# Autodesk Inventor assembly: carkifelek-ass
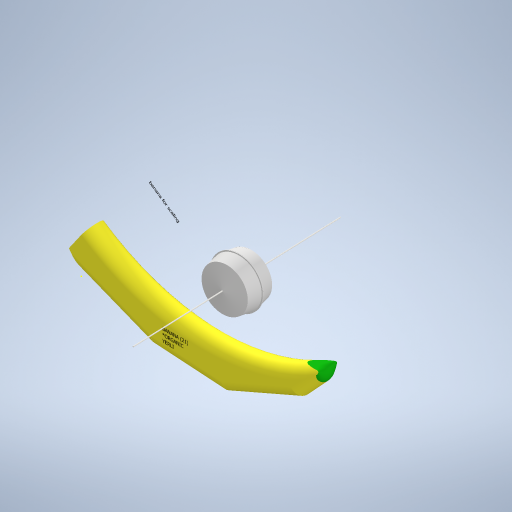
[picture p0: Inventor's stored thumbnail of the model, 512x512]
Saved by Autodesk Inventor 2023.2 (Build 272271000, 271)
## iProperties
Created: 2023-03-22
Part Number: carkifelek-ass
Document SubType Name: Assembly
Designer: sarp1
Author: sarp1
## Documents named in this file (7)
- C:\Users\sarp1\Documents\carkifelek-final\carkifelek-ass.iam
- C:\Users\sarp1\Documents\carkifelek-final\carkifelek-ass\Design Accelerator\Spur Gears1.iam
- C:\Users\sarp1\Documents\carkifelek-final\carkifelek-ass\Design Accelerator\Spur Gear11.ipt
- C:\Users\sarp1\Documents\carkifelek-final\dondurgec.ipt
- C:\Users\sarp1\Documents\carkifelek-final\carkifelek-ass\Design Accelerator\Spur Gear21.ipt
- C:\Users\sarp1\Documents\carkifelek-final\kab.ipt
- C:\Users\sarp1\Documents\carkifelek-final\scale.ipt
## Components (12 placed, 6 different names)
1. carks:1 [sub-assembly]
2. kucuk:1 — Cylindrical:2, Mate:5
3. dondurgec:1 — Cylindrical:1, Mate:1, Cylindrical:2, Cylindrical:3, Cylindrical:4, Cylindrical:5, Mate:3, Mate:4
4. boyuk:1 — Cylindrical:1, Mate:1, Cylindrical:11
5. kucuk:2 — Cylindrical:3, Mate:4
6. kucuk:3 — Cylindrical:4, Mate:3, Cylindrical:7
7. kucuk:4 — Cylindrical:5, Cylindrical:8, Mate:6
8. dondurgec:2 — Cylindrical:6, Mate:2, Cylindrical:7, Cylindrical:8, Mate:5, Mate:6
9. boyuk:2 — Cylindrical:6, Mate:2, Cylindrical:9, Cylindrical:10
10. kab:1 — Cylindrical:9, Cylindrical:10, Mate:7
11. kab:2 — Cylindrical:11, Mate:7
12. scale:1
## Relationships (18: CylindricalJoint 11, Mate 7)
- Cylindrical:1: dondurgec:1 ↔ boyuk:1
- Mate:1: dondurgec:1 ↔ boyuk:1
- Cylindrical:2: kucuk:1 ↔ dondurgec:1
- Cylindrical:3: dondurgec:1 ↔ kucuk:2
- Cylindrical:4: dondurgec:1 ↔ kucuk:3
- Cylindrical:5: dondurgec:1 ↔ kucuk:4
- Cylindrical:6: dondurgec:2 ↔ boyuk:2
- Mate:2: dondurgec:2 ↔ boyuk:2
- Mate:3: dondurgec:1 ↔ kucuk:3
- Mate:4: dondurgec:1 ↔ kucuk:2
- Cylindrical:7: kucuk:3 ↔ dondurgec:2
- Cylindrical:8: kucuk:4 ↔ dondurgec:2
- Mate:5: kucuk:1 ↔ dondurgec:2
- Mate:6: kucuk:4 ↔ dondurgec:2
- Cylindrical:9: boyuk:2 ↔ kab:1
- Cylindrical:10: boyuk:2 ↔ kab:1
- Cylindrical:11: boyuk:1 ↔ kab:2
- Mate:7: kab:1 ↔ kab:2
